# Autodesk Inventor assembly: Drive Gear Assembly
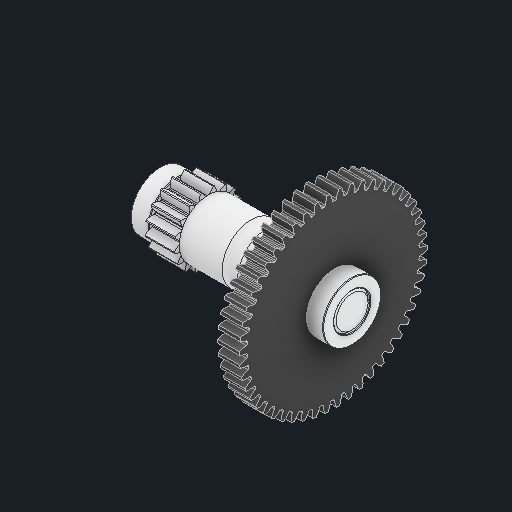
[picture p0: Inventor's stored thumbnail of the model, 512x512]
Saved by Autodesk Inventor 2025.1 (Build 291241020, 241B)
## iProperties
Created: 2025-05-11
Part Number: Drive Gear Assembly
Document SubType Name: Assembly
Designer: Joshua Eah
Author: Joshua Eah
## Documents named in this file (4)
- C:\Users\Joshua Eah\Documents\Voron 0.2\CAD\Master Assembly\Toolhead\Drive Gear Assembly.iam
- C:\Users\Joshua Eah\Documents\Voron 0.2\CAD\Master Assembly\MR85 Bearing.ipt
- C:\Users\Joshua Eah\Documents\Voron 0.2\CAD\Master Assembly\Drive Gear.ipt
- C:\Users\Joshua Eah\Documents\Voron 0.2\CAD\Master Assembly\Toolhead\50 Tooth Gear.ipt
## Components (4 placed, 3 different names)
1. MR85 Bearing:1 — Insert:2
2. Drive Gear:1 — Insert:3
3. 50 Tooth Gear:1 — Insert:1, Insert:2
4. MR85 Bearing:2 — Insert:1, Insert:3
## Relationships (3: Insert 3)
- Insert:1: 50 Tooth Gear:1 ↔ MR85 Bearing:2
- Insert:2: MR85 Bearing:1 ↔ 50 Tooth Gear:1
- Insert:3 (0.2 mm): Drive Gear:1 ↔ MR85 Bearing:2
